# Autodesk Inventor assembly: Robot Humanoid
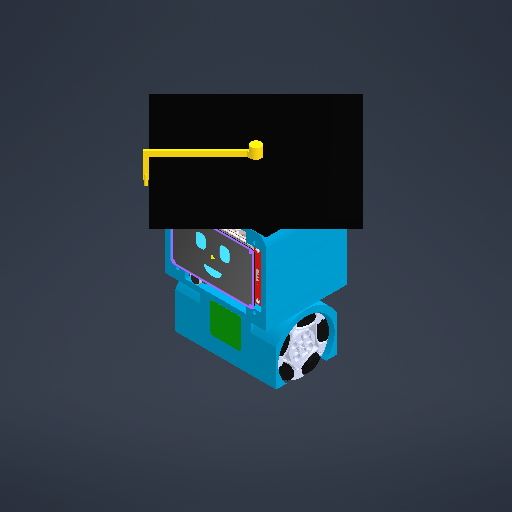
[picture p0: Inventor's stored thumbnail of the model, 512x512]
Saved by Autodesk Inventor 2026.2 (Build 302298000, 298)
## iProperties
Created: 2026-01-07
Part Number: Robot Humanoid
Document SubType Name: Assembly
Designer: hando
Author: hando
## Documents named in this file (18)
- D:\Data_Lokal\Kuliah\Tri Wahyu (22518241023)\Lomba Essay\FKMPI Fair Essay Competition\Design Humanoid\Robot Humanoid.iam
- D:\Data_Lokal\Kuliah\Tri Wahyu (22518241023)\Lomba Essay\FKMPI Fair Essay Competition\Design Humanoid\Base Kepala.ipt
- D:\Data_Lokal\Kuliah\Tri Wahyu (22518241023)\Lomba Essay\FKMPI Fair Essay Competition\2-8-inch-tft-lcd-module-1.snapshot.16\LCD_MSP2807_fusion\LCD_MSP2807_fusion\LCD_MSP2807_fusion.iam
- D:\Data_Lokal\Kuliah\Tri Wahyu (22518241023)\Lomba Essay\FKMPI Fair Essay Competition\esp-32-3.snapshot.1\ESP32\ESP32\ESP32.ipt
- D:\Data_Lokal\Kuliah\Tri Wahyu (22518241023)\Lomba Essay\FKMPI Fair Essay Competition\dfplayer-mini-3.snapshot.1\DFPlayer Mini Assem v1\DFPlayer Mini Assem v1\DFPlayer Mini Assem v1.iam
- D:\Data_Lokal\Kuliah\Tri Wahyu (22518241023)\Lomba Essay\FKMPI Fair Essay Competition\18650-retainers-1.snapshot.4\BK-18650-PC6\BK-18650-PC6\BK-18650-PC6.ipt
- D:\Data_Lokal\Kuliah\Tri Wahyu (22518241023)\Lomba Essay\FKMPI Fair Essay Competition\Design Humanoid\Tutup Baterai.ipt
- D:\Data_Lokal\Kuliah\Tri Wahyu (22518241023)\Lomba Essay\FKMPI Fair Essay Competition\usb-c-pd-board-zy12pdn-1.snapshot.2\USB-C PD board ZY12PDN\USB-C PD board ZY12PDN\USB-C PD board ZY12PDN.iam
- D:\Data_Lokal\Kuliah\Tri Wahyu (22518241023)\Lomba Essay\FKMPI Fair Essay Competition\speaker-2-inch-1.snapshot.1\Speaker 2 inch\Speaker 2 inch\Speaker 2 inch.ipt
- D:\Data_Lokal\Kuliah\Tri Wahyu (22518241023)\Lomba Essay\FKMPI Fair Essay Competition\analog-sound-sensor-microphone-module-1.snapshot.1\Microphone module\Microphone module\Microphone module.ipt
- D:\Data_Lokal\Kuliah\Tri Wahyu (22518241023)\Restek\Omni Base\Roda Omni_53mm.iam
- D:\Data_Lokal\Kuliah\Tri Wahyu (22518241023)\Lomba Essay\FKMPI Fair Essay Competition\motor\motor\motor.ipt
- D:\Data_Lokal\Kuliah\Tri Wahyu (22518241023)\Lomba Essay\FKMPI Fair Essay Competition\tb6612fng-driver-1.snapshot.2\SLDPRT\TB6612FNG_Upper Pins\TB6612FNG_Upper Pins\TB6612FNG_Upper Pins.ipt
- D:\Data_Lokal\Kuliah\Tri Wahyu (22518241023)\Lomba Essay\FKMPI Fair Essay Competition\capteur-gyroscopique-analogique-accelerometre-3-axes-mpu-6050-1.snapshot.2\MPU-6050\MPU-6050\MPU-6050\MPU-6050.iam
- D:\Data_Lokal\Kuliah\Tri Wahyu (22518241023)\Lomba Essay\FKMPI Fair Essay Competition\Design Humanoid\Skin KepalaV2.ipt
- D:\Data_Lokal\Kuliah\Tri Wahyu (22518241023)\Lomba Essay\FKMPI Fair Essay Competition\Design Humanoid\KacaLayar.ipt
- D:\Data_Lokal\Kuliah\Tri Wahyu (22518241023)\Lomba Essay\FKMPI Fair Essay Competition\Design Humanoid\TutupBawah.ipt
- D:\Data_Lokal\Kuliah\Tri Wahyu (22518241023)\Lomba Essay\FKMPI Fair Essay Competition\Design Humanoid\TobaCoba.ipt
## Components (20 placed, 17 different names)
1. Base Kepala:1 — Mate:2, Mate:3, Mate:5, Mate:6, Mate:8, Mate:12, Mate:13, Mate:14, Mate:15, Mate:23, Mate:24, Mate:25, Flush:1, Mate:26, Mate:27, Mate:29, Mate:30, Mate:31, Mate:34, Mate:35, Mate:36, Mate:37, Mate:38, Mate:39, Flush:2, Flush:3, Mate:44, Mate:45, Mate:49, Mate:50, Mate:51, Mate:52, Mate:53
2. LCD_MSP2807_fusion:1 [sub-assembly] — Mate:14, Mate:15
3. ESP32:1 — Mate:38, Mate:39
4. DFPlayer Mini Assem v1:1 [sub-assembly] — Mate:8, Mate:24
5. BK-18650-PC6:1 — Mate:2, Mate:3, Mate:25
6. Tutup Baterai:1 — Mate:5, Mate:6
7. USB-C PD board ZY12PDN:1 [sub-assembly] — Mate:12, Mate:13
8. Speaker 2 inch:1 — Mate:23, Mate:34, Mate:35
9. Microphone module:1 — Flush:1, Mate:26
10. Roda Omni_53mm:1 [sub-assembly] — Mate:42, Mate:43
11. Roda Omni_53mm:2 [sub-assembly] — Mate:40, Mate:41
12. motor:1 — Mate:27, Mate:29, Flush:3, Mate:40, Mate:41
13. motor:2 — Mate:30, Mate:31, Flush:2, Mate:42, Mate:43
14. TB6612FNG_Upper Pins:1 — Mate:36, Mate:37
15. MPU-6050:1 [sub-assembly] — Mate:44
16. Skin KepalaV2:1 — Mate:45, Mate:47, Mate:48, Mate:53, Mate:54, Mate:55
17. KacaLayar:1 — Mate:47, Mate:48
18. TutupBawah:1 — Mate:49, Mate:50
19. TutupBawah:2 — Mate:51, Mate:52
20. TobaCoba:1 — Mate:54, Mate:55
## Relationships (41: Mate 38, Flush 3)
- Mate:2: Base Kepala:1 ↔ BK-18650-PC6:1
- Mate:3: Base Kepala:1 ↔ BK-18650-PC6:1
- Mate:5: Base Kepala:1 ↔ Tutup Baterai:1
- Mate:6: Base Kepala:1 ↔ Tutup Baterai:1
- Mate:8 (10 mm): Base Kepala:1 ↔ DFPlayer Mini Assem v1:1
- Mate:12: Base Kepala:1 ↔ USB-C PD board ZY12PDN:1
- Mate:13 (2.5 mm): Base Kepala:1 ↔ USB-C PD board ZY12PDN:1
- Mate:14: Base Kepala:1 ↔ LCD_MSP2807_fusion:1
- Mate:15: Base Kepala:1 ↔ LCD_MSP2807_fusion:1
- Mate:23: Base Kepala:1 ↔ Speaker 2 inch:1
- Mate:24 (10 mm): Base Kepala:1 ↔ DFPlayer Mini Assem v1:1
- Mate:25: Base Kepala:1 ↔ BK-18650-PC6:1
- Flush:1: Base Kepala:1 ↔ Microphone module:1
- Mate:26: Base Kepala:1 ↔ Microphone module:1
- Mate:27: Base Kepala:1 ↔ motor:1
- Mate:29 (-1 mm): Base Kepala:1 ↔ motor:1
- Mate:30: Base Kepala:1 ↔ motor:2
- Mate:31 (-1 mm): Base Kepala:1 ↔ motor:2
- Mate:34: Base Kepala:1 ↔ Speaker 2 inch:1
- Mate:35: Base Kepala:1 ↔ Speaker 2 inch:1
- Mate:36 (2 mm): Base Kepala:1 ↔ TB6612FNG_Upper Pins:1
- Mate:37 (-40 mm): Base Kepala:1 ↔ TB6612FNG_Upper Pins:1
- Mate:38: Base Kepala:1 ↔ ESP32:1
- Mate:39 (18 mm): Base Kepala:1 ↔ ESP32:1
- Flush:2: Base Kepala:1 ↔ motor:2
- Flush:3: Base Kepala:1 ↔ motor:1
- Mate:40: Roda Omni_53mm:2 ↔ motor:1
- Mate:41 (3 mm): Roda Omni_53mm:2 ↔ motor:1
- Mate:42: Roda Omni_53mm:1 ↔ motor:2
- Mate:43 (3 mm): Roda Omni_53mm:1 ↔ motor:2
- Mate:44 (2 mm): Base Kepala:1 ↔ MPU-6050:1
- Mate:45: Base Kepala:1 ↔ Skin KepalaV2:1
- Mate:47: Skin KepalaV2:1 ↔ KacaLayar:1
- Mate:48: Skin KepalaV2:1 ↔ KacaLayar:1
- Mate:49: Base Kepala:1 ↔ TutupBawah:1
- Mate:50: Base Kepala:1 ↔ TutupBawah:1
- Mate:51: Base Kepala:1 ↔ TutupBawah:2
- Mate:52: Base Kepala:1 ↔ TutupBawah:2
- Mate:53: Base Kepala:1 ↔ Skin KepalaV2:1
- Mate:54: Skin KepalaV2:1 ↔ TobaCoba:1
- Mate:55: Skin KepalaV2:1 ↔ TobaCoba:1
